# Autodesk Inventor assembly: Assembly1
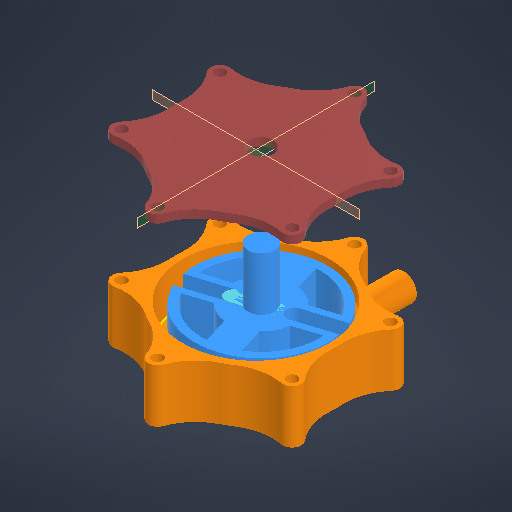
[picture p0: Inventor's stored thumbnail of the model, 512x512]
Saved by Autodesk Inventor 2025.3 (Build 293356000, 356)
## iProperties
Created: 2025-10-02
Part Number: Assembly1
Document SubType Name: Assembly
Designer: sophi
Author: sophi
## Documents named in this file (6)
- C:\Users\sophi\OneDrive - Universidad de los andes\Documentos\1 Universidad\5 Semestre\Herramientas\Huron-Hudson\Vane Engine\Vane\Assembly1.iam
- C:\Users\sophi\OneDrive - Universidad de los andes\Documentos\1 Universidad\5 Semestre\Herramientas\Huron-Hudson\Vane Engine\Vane\carcaza motor.ipt
- C:\Users\sophi\OneDrive - Universidad de los andes\Documentos\1 Universidad\5 Semestre\Herramientas\Huron-Hudson\Vane Engine\Vane\intermo.ipt
- C:\Users\sophi\OneDrive - Universidad de los andes\Documentos\1 Universidad\5 Semestre\Herramientas\Huron-Hudson\Vane Engine\Vane\paletas.ipt
- C:\Users\sophi\OneDrive - Universidad de los andes\Documentos\1 Universidad\5 Semestre\Herramientas\Huron-Hudson\Vane Engine\Vane\rodamiento.ipt
- C:\Users\sophi\OneDrive - Universidad de los andes\Documentos\1 Universidad\5 Semestre\Herramientas\Huron-Hudson\Vane Engine\Vane\tapa.ipt
## Components (6 placed, 5 different names)
1. carcaza motor:1 — Flush:1, Flush:2, Flush:3, Mate:9, Mate:10, Mate:16
2. intermo:1 — Mate:11, Mate:12, Mate:17
3. paletas:1 — Mate:12, Mate:13, Mate:15
4. rodamiento:1 — Mate:9, Mate:10, Mate:11, Mate:13, Mate:14
5. rodamiento:2 — Mate:14, Mate:15
6. tapa:1 — Mate:16, Mate:17
## Relationships (12: Mate 9, Flush 3)
- Flush:1: carcaza motor:1
- Flush:2: carcaza motor:1
- Flush:3: carcaza motor:1
- Mate:9: carcaza motor:1 ↔ rodamiento:1
- Mate:10: carcaza motor:1 ↔ rodamiento:1
- Mate:11: intermo:1 ↔ rodamiento:1
- Mate:12: intermo:1 ↔ paletas:1
- Mate:13: paletas:1 ↔ rodamiento:1
- Mate:14: rodamiento:1 ↔ rodamiento:2
- Mate:15: paletas:1 ↔ rodamiento:2
- Mate:16: carcaza motor:1 ↔ tapa:1
- Mate:17: intermo:1 ↔ tapa:1
